# Autodesk Inventor assembly: 42146-05
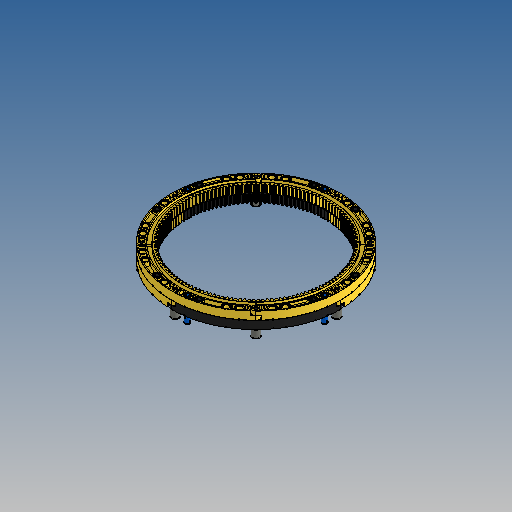
[picture p0: Inventor's stored thumbnail of the model, 512x512]
Saved by Autodesk Inventor 2025 (Build 290162010, 162A)
## iProperties
Created: 2024-11-14
Part Number: 42146-05
Material: Generisch
Document SubType Name: Assembly
Designer: hp.muther
Author: hp.muther
## Documents named in this file (7)
- D:\Inventor\Projekte\Muther\LEGO Technic\LEGO Technik - Raupenkran LR 13000 (42146)\42146-01-05.iam
- D:\Inventor\Projekte\Muther\LEGO Technic\LEGO Pieces\Zahnrad\24121-Black.ipt
- D:\Inventor\Projekte\Muther\LEGO Technic\LEGO Pieces\Pin's\18651-Black.ipt
- D:\Inventor\Projekte\Muther\LEGO Technic\LEGO Pieces\Rund\18654-DkBluishGray.ipt
- D:\Inventor\Projekte\Muther\LEGO Technic\LEGO Pieces\Zahnrad\24121-Yellow.ipt
- D:\Inventor\Projekte\Muther\LEGO Technic\LEGO Pieces\Pin's\2780-Black.ipt
- D:\Inventor\Projekte\Muther\LEGO Technic\LEGO Pieces\Pin's\6558-Blue.ipt
## Components (36 placed, 6 different names)
1. 24121-Black:1 — Einfügen:1, Einfügen:5, Einfügen:6, Einfügen:8, Passend:1, Einfügen:12, Passend:4, Einfügen:29, Einfügen:30, Passend:9, Einfügen:34, Einfügen:35
2. 18651-Black:1 — Einfügen:1, Einfügen:2, Passend:9, Passend:11
3. 18654-DkBluishGray:1 — Einfügen:2
4. 18651-Black:2 — Einfügen:5
5. 18654-DkBluishGray:2
6. 18651-Black:3 — Einfügen:6
7. 18654-DkBluishGray:3
8. 18651-Black:4 — Einfügen:9, Passend:2
9. 18654-DkBluishGray:4
10. 24121-Yellow:1 — Einfügen:8, Passend:1, Einfügen:9, Passend:2, Einfügen:19, Einfügen:27, Einfügen:28
11. 18651-Black:5
12. 18654-DkBluishGray:5
13. 24121-Yellow:2 — Einfügen:12, Passend:4, Passend:5, Einfügen:23, Einfügen:24
14. 24121-Black:2 — Einfügen:19, Passend:5, Einfügen:25, Einfügen:26, Passend:10, Einfügen:31, Einfügen:32, Einfügen:33
15. 18651-Black:6 — Passend:10
16. 18654-DkBluishGray:6
17. 18651-Black:7
18. 18654-DkBluishGray:7
19. 18651-Black:8
20. 18654-DkBluishGray:8
21. 24121-Yellow:6 — Passend:11
22. 24121-Yellow:3
23. 24121-Yellow:4 — Einfügen:31
24. 24121-Yellow:5
25. 2780-Black:1 — Einfügen:26
26. 2780-Black:2 — Einfügen:24
27. 2780-Black:3 — Einfügen:25
28. 2780-Black:4 — Einfügen:28
29. 2780-Black:5 — Einfügen:27
30. 2780-Black:6 — Einfügen:23
31. 2780-Black:7 — Einfügen:29
32. 2780-Black:8 — Einfügen:30
33. 6558-Blue:1 — Einfügen:35
34. 6558-Blue:2 — Einfügen:33
35. 6558-Blue:3 — Einfügen:32
36. 6558-Blue:4 — Einfügen:34
## Relationships (46: Insert 35, Mate 11)
- Einfügen:1 [Insert]: 24121-Black:1 ↔ 18651-Black:1
- Einfügen:2 [Insert]: 18651-Black:1 ↔ 18654-DkBluishGray:1
- [Insert]: 18651-Black:2 ↔ 18654-DkBluishGray:2
- [Insert]: 18651-Black:3 ↔ 18654-DkBluishGray:3
- Einfügen:5 [Insert]: 24121-Black:1 ↔ 18651-Black:2
- Einfügen:6 [Insert]: 24121-Black:1 ↔ 18651-Black:3
- [Insert]: 18651-Black:4 ↔ 18654-DkBluishGray:4
- Einfügen:8 [Insert]: 24121-Black:1 ↔ 24121-Yellow:1
- Passend:1 [Mate]: 24121-Black:1 ↔ 24121-Yellow:1
- Einfügen:9 [Insert]: 18651-Black:4 ↔ 24121-Yellow:1
- Passend:2 [Mate]: 18651-Black:4 ↔ 24121-Yellow:1
- [Insert]: 18651-Black:5 ↔ 18654-DkBluishGray:5
- [Insert]: 18651-Black:5 ↔ 24121-Yellow:2
- [Mate]: 18651-Black:5 ↔ 24121-Yellow:2
- Einfügen:12 [Insert]: 24121-Black:1 ↔ 24121-Yellow:2
- Passend:4 [Mate]: 24121-Black:1 ↔ 24121-Yellow:2
- [Insert]: 24121-Black:2 ↔ 18651-Black:6
- [Insert]: 18651-Black:6 ↔ 18654-DkBluishGray:6
- [Insert]: 18651-Black:7 ↔ 18654-DkBluishGray:7
- [Insert]: 18651-Black:8 ↔ 18654-DkBluishGray:8
- [Insert]: 24121-Black:2 ↔ 18651-Black:7
- [Insert]: 24121-Black:2 ↔ 18651-Black:8
- Einfügen:19 [Insert]: 24121-Yellow:1 ↔ 24121-Black:2
- Passend:5 [Mate]: 24121-Yellow:2 ↔ 24121-Black:2
- [Insert]: 24121-Yellow:6 ↔ 24121-Yellow:3
- [Mate]: 24121-Yellow:6 ↔ 24121-Yellow:3
- [Insert]: 24121-Yellow:6 ↔ 24121-Yellow:4
- [Mate]: 24121-Yellow:6 ↔ 24121-Yellow:4
- [Insert]: 24121-Yellow:3 ↔ 24121-Yellow:5
- [Mate]: 24121-Yellow:4 ↔ 24121-Yellow:5
- Einfügen:23 [Insert]: 24121-Yellow:2 ↔ 2780-Black:6
- Einfügen:24 [Insert]: 24121-Yellow:2 ↔ 2780-Black:2
- Einfügen:25 [Insert]: 24121-Black:2 ↔ 2780-Black:3
- Einfügen:26 [Insert]: 24121-Black:2 ↔ 2780-Black:1
- Einfügen:27 [Insert]: 24121-Yellow:1 ↔ 2780-Black:5
- Einfügen:28 [Insert]: 24121-Yellow:1 ↔ 2780-Black:4
- Einfügen:29 [Insert]: 24121-Black:1 ↔ 2780-Black:7
- Einfügen:30 [Insert]: 24121-Black:1 ↔ 2780-Black:8
- Passend:9 [Mate]: 24121-Black:1 ↔ 18651-Black:1
- Passend:10 [Mate]: 24121-Black:2 ↔ 18651-Black:6
- Einfügen:31 [Insert]: 24121-Black:2 ↔ 24121-Yellow:4
- Passend:11 [Mate]: 18651-Black:1 ↔ 24121-Yellow:6
- Einfügen:32 [Insert]: 24121-Black:2 ↔ 6558-Blue:3
- Einfügen:33 [Insert]: 24121-Black:2 ↔ 6558-Blue:2
- Einfügen:34 [Insert]: 24121-Black:1 ↔ 6558-Blue:4
- Einfügen:35 [Insert]: 24121-Black:1 ↔ 6558-Blue:1
## Named parameters: d2_d1 = 0 mm, d3_d1 = 0 mm, d6_d3_d1 = 0 mm, d11_d6_d3_d1 = 0 mm, d12_d9 = 0 mm, d13_d10 = 0 mm, d16_d0 = 0 mm, d17_d1 = 0 mm, d18_d2_d1 = 0 mm, d19_d3_d1 = 0 mm, d20_d4 = 0 mm, d21_d5 = 0 mm, d24_d7 = 0 mm, d25_d8 = 0 mm, d26_d14 = 0 mm, d27_d15 = 0 mm, d28_d22 = 0 mm, d29_d23 = 0 mm
